# Autodesk Inventor assembly: FEICHAO BE4108 380KV
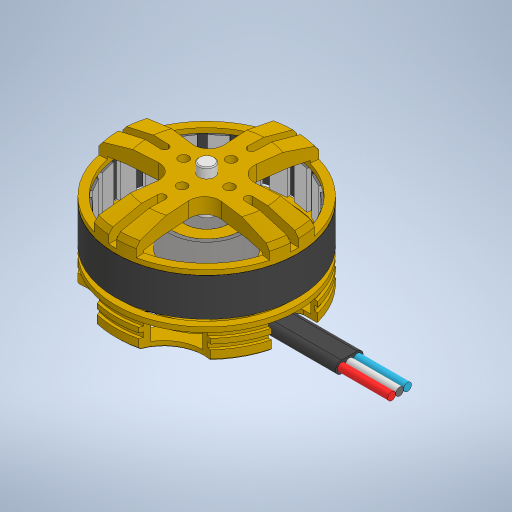
[picture p0: Inventor's stored thumbnail of the model, 512x512]
Saved by Autodesk Inventor 2023.4 (Build 274418000, 418)
## iProperties
Created: 2022-11-08
Part Number: FEICHAO BE4108 380KV
Document SubType Name: Assembly
Designer: Nathan Cai
Mass: 113 g
Surface Area: 168.17 cm^2
Volume: 12.8283 cm^3
Author: Nathan Cai
## Documents named in this file (7)
- E:\Documents\Inventor\Law - V2.1\Vert - Basic\FEICHAO BE4108 380KV\FEICHAO BE4108 380KV.iam
- E:\Documents\Inventor\Law - V2.1\FEICHAO BE4108 380KV\BASE.ipt
- E:\Documents\Inventor\Law - V2.1\FEICHAO BE4108 380KV\METAL RING.ipt
- E:\Documents\Inventor\Law - V2.1\FEICHAO BE4108 380KV\SHAFT.ipt
- E:\Documents\Inventor\Law - V2.1\FEICHAO BE4108 380KV\CAN.ipt
- E:\Documents\Inventor\Law - V2.1\FEICHAO BE4108 380KV\BEARING.ipt
- E:\Documents\Inventor\Law - V2.1\FEICHAO BE4108 380KV\CABLE.ipt
## Components (7 placed, 6 different names)
1. BASE:1 — Mate:1, Flush:1, Mate:2, Mate:4, Mate:5, Flush:3, Flush:4, Flush:5, Tangent:1, Mate:7
2. METAL RING:1 — Mate:1, Flush:1
3. SHAFT:1 — Mate:2, Mate:3, Flush:2, Mate:6
4. CAN:1 — Mate:3, Flush:2, Mate:4
5. BEARING:1 — Mate:5, Flush:3
6. BEARING:2 — Mate:6, Flush:4
7. CABLE:1 — Flush:5, Tangent:1, Mate:7
## Relationships (13: Mate 7, Flush 5, Tangent 1)
- Mate:1: BASE:1 ↔ METAL RING:1
- Flush:1: BASE:1 ↔ METAL RING:1
- Mate:2: BASE:1 ↔ SHAFT:1
- Mate:3: SHAFT:1 ↔ CAN:1
- Flush:2 (2.5 mm): SHAFT:1 ↔ CAN:1
- Mate:4 (-25 mm): BASE:1 ↔ CAN:1
- Mate:5: BASE:1 ↔ BEARING:1
- Flush:3: BASE:1 ↔ BEARING:1
- Mate:6: SHAFT:1 ↔ BEARING:2
- Flush:4: BASE:1 ↔ BEARING:2
- Flush:5: BASE:1 ↔ CABLE:1
- Tangent:1: BASE:1 ↔ CABLE:1
- Mate:7: BASE:1 ↔ CABLE:1
